# Autodesk Inventor assembly: 16in 8020
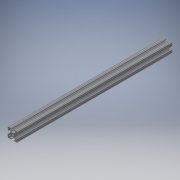
[picture p0: Inventor's stored thumbnail of the model, 180x180]
Saved by Autodesk Inventor 2019 (Build 230136000, 136)
## iProperties
Created: 2019-01-18
Part Number: 16in 8020
Document SubType Name: Assembly
Designer: Tiberus
Author: Tiberus
## Documents named in this file (2)
- G:\Robotics\Ball Intake 2019\16in 8020.iam
- G:\Robotics\Ball Intake 2019\10_Series\10_Series\1010.IPT
## Components (2 placed, 1 different names)
1. 1010:1 — Mate:1, Flush:1, Flush:2
2. 1010:2 — Mate:1, Flush:1, Flush:2
## Relationships (3: Flush 2, Mate 1)
- Mate:1: 1010:1 ↔ 1010:2
- Flush:1: 1010:1 ↔ 1010:2
- Flush:2: 1010:1 ↔ 1010:2
